# Autodesk Inventor assembly: Joint Assembly
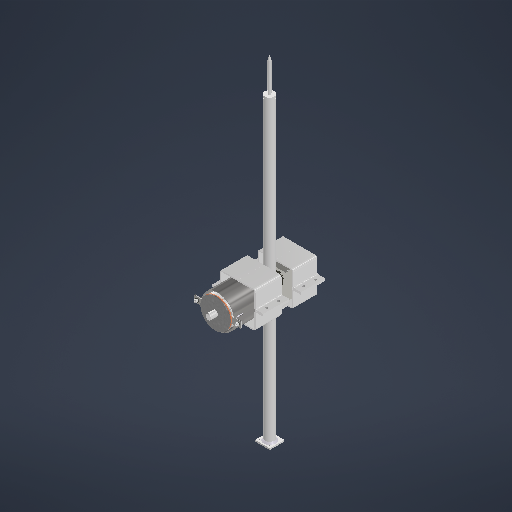
[picture p0: Inventor's stored thumbnail of the model, 512x512]
Saved by Autodesk Inventor 2026.3 (Build 303398000, 398)
## iProperties
Created: 2026-07-22
Part Number: Joint Assembly
Document SubType Name: Assembly
Designer: matot
Author: matot
## Documents named in this file (15)
- C:\Users\matot\OneDrive - Stellenbosch University\2026\MechatronicsProject478\Building the joint\Joint Assembly\Joint Assembly.iam
- C:\Users\matot\OneDrive - Stellenbosch University\2026\MechatronicsProject478\Building the joint\Joint Assembly\Final joint shaft.ipt
- C:\Users\matot\OneDrive - Stellenbosch University\2026\MechatronicsProject478\Building the joint\Joint Assembly\2058786.iam
- C:\Users\matot\OneDrive - Stellenbosch University\2026\MechatronicsProject478\Building the joint\Joint Assembly\8236967.ipt
- C:\Users\matot\OneDrive - Stellenbosch University\2026\MechatronicsProject478\Building the joint\Joint Assembly\Optical Encoder.ipt
- C:\Users\matot\OneDrive - Stellenbosch University\2026\MechatronicsProject478\Building the joint\Joint Assembly\Brake disc.ipt
- C:\Users\matot\OneDrive - Stellenbosch University\2026\MechatronicsProject478\Building the joint\Joint Assembly\Bearing housing top.ipt
- C:\Users\matot\OneDrive - Stellenbosch University\2026\MechatronicsProject478\Building the joint\Joint Assembly\Bearing housing bottom.ipt
- C:\Users\matot\OneDrive - Stellenbosch University\2026\MechatronicsProject478\Building the joint\Joint Assembly\Joint Housing Bottom_final.iam
- C:\Users\matot\OneDrive - Stellenbosch University\2026\MechatronicsProject478\Building the joint\Joint Assembly\Complete front top housing.iam
- C:\Users\matot\OneDrive - Stellenbosch University\2026\MechatronicsProject478\Building the joint\Joint Assembly\Complete back top housing.iam
- C:\Users\matot\OneDrive - Stellenbosch University\2026\MechatronicsProject478\Building the joint\Joint Assembly\Base link.iam
- C:\Users\matot\OneDrive - Stellenbosch University\2026\MechatronicsProject478\Building the joint\Joint Assembly\Output Link.iam
- C:\Users\matot\OneDrive - Stellenbosch University\2026\MechatronicsProject478\Building the joint\Joint Assembly\Key.ipt
- C:\Users\matot\OneDrive - Stellenbosch University\2026\MechatronicsProject478\Building the joint\Joint Assembly\Electromanetic brake.iam
## Components (18 placed, 14 different names)
1. Final joint shaft:1 — Insert:1, Insert:2, Mate:1, Insert:5, Tangent:3, Mate:17, Tangent:4, Mate:24, Mate:25, Flush:19, Mate:26
2. 2058786:1 [sub-assembly] — Insert:2, Insert:4, Insert:17, Insert:20
3. 2058786:2 [sub-assembly] — Insert:1, Insert:3, Insert:18, Insert:19
4. 8236967:1 — Insert:4
5. 8236967:2 — Insert:3
6. Optical Encoder:1 — Mate:1, Insert:5
7. Bearing housing top:1 — Insert:17, Mate:14
8. Bearing housing top:2 — Insert:18, Mate:13
9. Bearing housing bottom:1 — Insert:20, Mate:14, Mate:15
10. Bearing housing bottom:2 — Insert:19, Mate:13, Mate:16
11. Joint Housing Bottom_final:2 [sub-assembly] — Mate:11, Flush:11, Flush:12, Flush:13, Mate:12, Flush:14, Mate:15, Mate:16, Insert:21, Insert:22
12. Complete front top housing:1 [sub-assembly] — Mate:11, Flush:11, Flush:12, Tangent:5
13. Complete back top housing:1 [sub-assembly] — Flush:13, Mate:12, Flush:14
14. Base link:1 [sub-assembly] — Insert:21, Insert:22
15. Output Link:1 [sub-assembly] — Tangent:3, Mate:17, Tangent:4
16. Key:1 — Mate:24, Mate:25, Flush:19, Mate:27, Mate:28, Mate:30
17. Electromanetic brake:1 [sub-assembly] — Mate:26, Mate:27, Tangent:5, Mate:29
18. Brake disc:1 — Mate:28, Mate:29, Mate:30
## Relationships (34: Mate 15, Insert 11, Flush 5, Tangent 3)
- Insert:1: Final joint shaft:1 ↔ 2058786:2
- Insert:2: Final joint shaft:1 ↔ 2058786:1
- Insert:3: 2058786:2 ↔ 8236967:2
- Insert:4: 2058786:1 ↔ 8236967:1
- Mate:1: Final joint shaft:1 ↔ Optical Encoder:1
- Insert:5: Final joint shaft:1 ↔ Optical Encoder:1
- Insert:17: 2058786:1 ↔ Bearing housing top:1
- Insert:18: 2058786:2 ↔ Bearing housing top:2
- Insert:19: 2058786:2 ↔ Bearing housing bottom:2
- Insert:20: 2058786:1 ↔ Bearing housing bottom:1
- Mate:11: Joint Housing Bottom_final:2 ↔ Complete front top housing:1
- Flush:11: Joint Housing Bottom_final:2 ↔ Complete front top housing:1
- Flush:12: Joint Housing Bottom_final:2 ↔ Complete front top housing:1
- Flush:13: Joint Housing Bottom_final:2 ↔ Complete back top housing:1
- Mate:12: Joint Housing Bottom_final:2 ↔ Complete back top housing:1
- Flush:14: Joint Housing Bottom_final:2 ↔ Complete back top housing:1
- Mate:13: Bearing housing top:2 ↔ Bearing housing bottom:2
- Mate:14: Bearing housing top:1 ↔ Bearing housing bottom:1
- Mate:15: Bearing housing bottom:1 ↔ Joint Housing Bottom_final:2
- Mate:16: Bearing housing bottom:2 ↔ Joint Housing Bottom_final:2
- Insert:21: Joint Housing Bottom_final:2 ↔ Base link:1
- Insert:22: Joint Housing Bottom_final:2 ↔ Base link:1
- Tangent:3: Final joint shaft:1 ↔ Output Link:1
- Mate:17: Final joint shaft:1 ↔ Output Link:1
- Tangent:4: Final joint shaft:1 ↔ Output Link:1
- Mate:24: Final joint shaft:1 ↔ Key:1
- Mate:25: Final joint shaft:1 ↔ Key:1
- Flush:19: Final joint shaft:1 ↔ Key:1
- Mate:26: Final joint shaft:1 ↔ Electromanetic brake:1
- Mate:27: Key:1 ↔ Electromanetic brake:1
- Tangent:5: Complete front top housing:1 ↔ Electromanetic brake:1
- Mate:28: Key:1 ↔ Brake disc:1
- Mate:29 (1 mm): Electromanetic brake:1 ↔ Brake disc:1
- Mate:30: Key:1 ↔ Brake disc:1
